# Autodesk Inventor assembly: Bikair
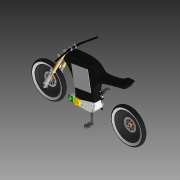
[picture p0: Inventor's stored thumbnail of the model, 180x180]
Saved by Autodesk Inventor 2016 (Build 200138000, 138)
## iProperties
Created: 2015-03-25
Part Number: Bikair
Document SubType Name: Assembly
Designer: Yann
Author: Yann
## Documents named in this file (11)
- C:\Users\Yann\Documents\GitHub\BIKAIR_CAD\Source\Bikair.iam
- C:\Users\Yann\Documents\GitHub\BIKAIR_CAD\Source\Frame\Frame.iam
- C:\Users\Yann\Documents\GitHub\BIKAIR_CAD\Source\Energy_Pack\Energy_Pack.iam
- C:\Users\Yann\Documents\GitHub\BIKAIR_CAD\Source\Motor\Motor.iam
- C:\Users\Yann\Documents\GitHub\BIKAIR_CAD\Source\Rear_Train\Rear_Train.iam
- C:\Users\Yann\Documents\GitHub\BIKAIR_CAD\Source\Rear_Train\Wheel\wheel.iam
- C:\Users\Yann\Documents\GitHub\BIKAIR_CAD\Source\Front_Train\Front_Train.iam
- C:\Users\Yann\Documents\GitHub\BIKAIR_CAD\Source\Bike_Drive\Bike_Drive.iam
- C:\Users\Yann\Documents\GitHub\BIKAIR_CAD\Source\Motor\Colossus_7kW.iam
- C:\Users\Yann\Documents\GitHub\BIKAIR_CAD\Source\Body\Shell.ipt
- C:\Users\Yann\Documents\GitHub\BIKAIR_CAD\Source\Shell\Shell.iam
## Components (13 placed, 9 different names)
1. Frame:1 [sub-assembly] — Affleurement:1, Placage:1, Placage:2, Mate:13, Flush:16
2. Energy_Pack:1 [sub-assembly] — Affleurement:2, Angle:1, Mate:11, Flush:13, Flush:14
3. Motor:1 [sub-assembly] — Placage:3
4. Rear_Train:1 [sub-assembly] — Affleurement:7
5. wheel:1 [sub-assembly] — Affleurement:5
6. wheel:3 [sub-assembly]
7. Front_Train:1 [sub-assembly] — Placage:5, Affleurement:8, Angle:4
8. Motor:2 [sub-assembly] — Placage:6
9. Bike_Drive:1 [sub-assembly] — Mate:13, Flush:16
10. Colossus_7kW:1 [sub-assembly]
11. Shell:1 — Flush:10, Flush:11, Flush:12
12. Energy_Pack:2 [sub-assembly] — Mate:11, Flush:13, Flush:14
13. Shell:2 [sub-assembly] — Flush:15
## Relationships (21: Flush 12, Mate 7, Angle 2)
- Affleurement:1 [Flush]: Frame:1
- Placage:1 [Mate]: Frame:1
- Placage:2 [Mate]: Frame:1
- Affleurement:2 [Flush] (-38 mm): Energy_Pack:1
- Angle:1 (10 deg): Energy_Pack:1
- Placage:3 [Mate] (40 mm): Motor:1
- Affleurement:5 [Flush]: wheel:1
- Affleurement:7 [Flush]: Rear_Train:1
- Placage:5 [Mate]: Front_Train:1
- Affleurement:8 [Flush]: Front_Train:1
- Angle:4 (25 deg): Front_Train:1
- Placage:6 [Mate]: Motor:2
- Flush:10: Shell:1
- Flush:11: Shell:1
- Flush:12: Shell:1
- Mate:11 (5 mm): Energy_Pack:1 ↔ Energy_Pack:2
- Flush:13: Energy_Pack:1 ↔ Energy_Pack:2
- Flush:14: Energy_Pack:1 ↔ Energy_Pack:2
- Flush:15: Shell:2
- Mate:13: Frame:1 ↔ Bike_Drive:1
- Flush:16 (10 mm): Frame:1 ↔ Bike_Drive:1
